# Autodesk Inventor assembly: Main-Assembly
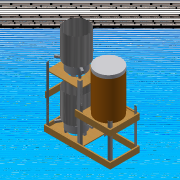
[picture p0: Inventor's stored thumbnail of the model, 180x180]
Saved by Autodesk Inventor 2017 (Build 210142000, 142)
## iProperties
Created: 2017-08-30
Part Number: Main-Assembly
Document SubType Name: Assembly
Designer: Trent
Author: Trent
## Documents named in this file (11)
- Z:\Users\trentshumay\Dev\IoT-GIT\brewing-rack\models\Main-Assembly.iam
- Z:\Users\trentshumay\Dev\IoT-GIT\brewing-rack\models\Kettle-Placeholder.ipt
- Z:\Users\trentshumay\Dev\IoT-GIT\brewing-rack\models\Tun-Placeholder.ipt
- Z:\Users\trentshumay\Dev\IoT-GIT\brewing-rack\models\36-inch-L.ipt
- Z:\Users\trentshumay\Dev\IoT-GIT\brewing-rack\models\Tun-Platform.ipt
- Z:\Users\trentshumay\Dev\IoT-GIT\brewing-rack\models\24-inch-L.ipt
- Z:\Users\trentshumay\Dev\IoT-GIT\brewing-rack\models\Kettle-Platform.ipt
- Z:\Users\trentshumay\Dev\IoT-GIT\brewing-rack\models\Burner-Placeholder.ipt
- Z:\Users\trentshumay\Dev\IoT-GIT\brewing-rack\models\Long-Brace.ipt
- Z:\Users\trentshumay\Dev\IoT-GIT\brewing-rack\models\Short-Brace.ipt
- Z:\Users\trentshumay\Dev\IoT-GIT\brewing-rack\models\Tun-Brace.ipt
## Components (24 placed, 10 different names)
1. Kettle-Placeholder:1 — Mate:16, Mate:17, Mate:33
2. Tun-Placeholder:1 — Mate:1, Flush:1, Flush:3, Flush:4, Flush:5
3. 36-inch-L:1 — Mate:10, Flush:10, Flush:11, Mate:12, Mate:13, Flush:15, Flush:17, Flush:19, Flush:20
4. Tun-Platform:1 — Mate:1, Flush:1, Flush:3, Flush:4, Flush:5, Mate:2, Mate:3, Flush:6, Mate:4, Mate:5, Mate:6, Mate:7, Mate:8, Mate:9
5. 24-inch-L:1 — Mate:2, Mate:3, Flush:6, Flush:7, Flush:9, Flush:25
6. 24-inch-L:2 — Mate:4, Mate:5, Flush:7, Flush:8, Flush:21, Mate:24
7. 24-inch-L:3 — Mate:8, Mate:9, Flush:9, Mate:11, Flush:12, Flush:13
8. 24-inch-L:4 — Mate:6, Mate:7, Flush:8, Mate:10, Flush:10, Flush:11
9. 36-inch-L:2 — Mate:11, Flush:12, Flush:13, Flush:16, Flush:18, Mate:19
10. 36-inch-L:3 — Flush:16, Mate:14, Flush:18, Mate:18, Mate:25, Mate:26
11. 36-inch-L:4 — Flush:17, Mate:15, Flush:19, Flush:22
12. Kettle-Platform:1 — Mate:12, Mate:13, Flush:15, Mate:14, Mate:15, Mate:16, Mate:17, Mate:34
13. Kettle-Platform:2 — Mate:18, Mate:19, Flush:20, Mate:20, Mate:21
14. Burner-Placeholder:1 — Mate:20, Mate:21, Mate:22, Mate:23
15. Kettle-Placeholder:2 — Mate:22, Mate:23
16. Long-Brace:1 — Flush:21, Mate:24, Flush:22, Flush:23, Flush:24, Flush:26, Flush:27, Mate:27, Flush:33, Flush:34
17. Long-Brace:2 — Mate:25, Flush:23, Flush:24, Flush:28, Mate:31
18. Long-Brace:3 — Flush:25, Flush:26, Mate:26, Flush:29, Flush:30, Mate:28, Flush:31, Mate:29, Flush:32
19. Short-Brace:1 — Flush:27, Flush:28, Mate:27
20. Short-Brace:2 — Flush:29, Flush:30, Mate:28, Mate:32, Flush:35, Flush:36
21. Short-Brace:3 — Flush:31, Mate:29, Flush:32
22. Short-Brace:4 — Flush:33, Mate:31, Flush:34
23. Tun-Brace:1 — Mate:32, Flush:35, Flush:36
24. Burner-Placeholder:2 — Mate:33, Mate:34
## Relationships (67: Flush 34, Mate 33)
- Mate:1: Tun-Placeholder:1 ↔ Tun-Platform:1
- Flush:1: Tun-Placeholder:1 ↔ Tun-Platform:1
- Flush:3 (38.1 mm): Tun-Placeholder:1 ↔ Tun-Platform:1
- Flush:4: Tun-Placeholder:1 ↔ Tun-Platform:1
- Flush:5 (12.7 mm): Tun-Placeholder:1 ↔ Tun-Platform:1
- Mate:2: Tun-Platform:1 ↔ 24-inch-L:1
- Mate:3: Tun-Platform:1 ↔ 24-inch-L:1
- Flush:6 (-101.6 mm): Tun-Platform:1 ↔ 24-inch-L:1
- Mate:4: Tun-Platform:1 ↔ 24-inch-L:2
- Mate:5: Tun-Platform:1 ↔ 24-inch-L:2
- Flush:7: 24-inch-L:1 ↔ 24-inch-L:2
- Mate:6: Tun-Platform:1 ↔ 24-inch-L:4
- Mate:7: Tun-Platform:1 ↔ 24-inch-L:4
- Flush:8: 24-inch-L:2 ↔ 24-inch-L:4
- Mate:8: Tun-Platform:1 ↔ 24-inch-L:3
- Mate:9: Tun-Platform:1 ↔ 24-inch-L:3
- Flush:9: 24-inch-L:1 ↔ 24-inch-L:3
- Mate:10: 36-inch-L:1 ↔ 24-inch-L:4
- Flush:10: 36-inch-L:1 ↔ 24-inch-L:4
- Flush:11: 36-inch-L:1 ↔ 24-inch-L:4
- Mate:11: 24-inch-L:3 ↔ 36-inch-L:2
- Flush:12: 24-inch-L:3 ↔ 36-inch-L:2
- Flush:13: 24-inch-L:3 ↔ 36-inch-L:2
- Mate:12: 36-inch-L:1 ↔ Kettle-Platform:1
- Mate:13: 36-inch-L:1 ↔ Kettle-Platform:1
- Flush:15 (25.4 mm): 36-inch-L:1 ↔ Kettle-Platform:1
- Flush:16: 36-inch-L:2 ↔ 36-inch-L:3
- Mate:14: 36-inch-L:3 ↔ Kettle-Platform:1
- Flush:17: 36-inch-L:1 ↔ 36-inch-L:4
- Mate:15: 36-inch-L:4 ↔ Kettle-Platform:1
- Flush:18: 36-inch-L:2 ↔ 36-inch-L:3
- Flush:19: 36-inch-L:1 ↔ 36-inch-L:4
- Mate:16: Kettle-Placeholder:1 ↔ Kettle-Platform:1
- Mate:17 (177.8 mm): Kettle-Placeholder:1 ↔ Kettle-Platform:1
- Mate:18: 36-inch-L:3 ↔ Kettle-Platform:2
- Mate:19: 36-inch-L:2 ↔ Kettle-Platform:2
- Flush:20 (101.6 mm): 36-inch-L:1 ↔ Kettle-Platform:2
- Mate:20: Kettle-Platform:2 ↔ Burner-Placeholder:1
- Mate:21: Kettle-Platform:2 ↔ Burner-Placeholder:1
- Mate:22: Burner-Placeholder:1 ↔ Kettle-Placeholder:2
- Mate:23: Burner-Placeholder:1 ↔ Kettle-Placeholder:2
- Flush:21 (-19.05 mm): 24-inch-L:2 ↔ Long-Brace:1
- Mate:24: 24-inch-L:2 ↔ Long-Brace:1
- Flush:22: 36-inch-L:4 ↔ Long-Brace:1
- Mate:25: 36-inch-L:3 ↔ Long-Brace:2
- Flush:23: Long-Brace:1 ↔ Long-Brace:2
- Flush:24: Long-Brace:1 ↔ Long-Brace:2
- Flush:25 (-88.9 mm): 24-inch-L:1 ↔ Long-Brace:3
- Flush:26: Long-Brace:1 ↔ Long-Brace:3
- Mate:26: 36-inch-L:3 ↔ Long-Brace:3
- Flush:27: Long-Brace:1 ↔ Short-Brace:1
- Flush:28: Long-Brace:2 ↔ Short-Brace:1
- Mate:27: Long-Brace:1 ↔ Short-Brace:1
- Flush:29: Long-Brace:3 ↔ Short-Brace:2
- Flush:30: Long-Brace:3 ↔ Short-Brace:2
- Mate:28: Long-Brace:3 ↔ Short-Brace:2
- Flush:31: Long-Brace:3 ↔ Short-Brace:3
- Mate:29: Long-Brace:3 ↔ Short-Brace:3
- Flush:32: Long-Brace:3 ↔ Short-Brace:3
- Flush:33: Long-Brace:1 ↔ Short-Brace:4
- Mate:31: Long-Brace:2 ↔ Short-Brace:4
- Flush:34: Long-Brace:1 ↔ Short-Brace:4
- Mate:32: Short-Brace:2 ↔ Tun-Brace:1
- Flush:35: Short-Brace:2 ↔ Tun-Brace:1
- Flush:36: Short-Brace:2 ↔ Tun-Brace:1
- Mate:33: Kettle-Placeholder:1 ↔ Burner-Placeholder:2
- Mate:34: Kettle-Platform:1 ↔ Burner-Placeholder:2
